# Autodesk Inventor assembly: EL2-.200
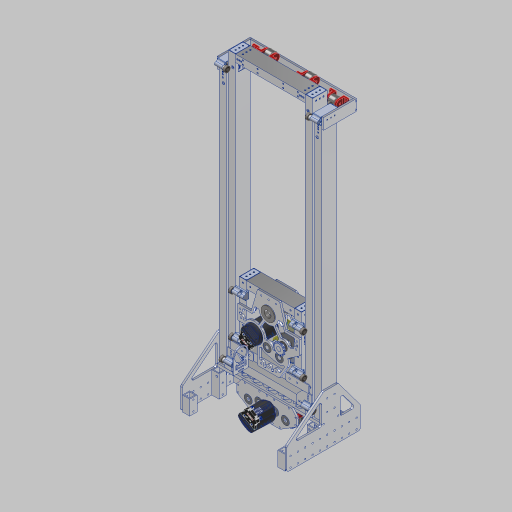
[picture p0: Inventor's stored thumbnail of the model, 512x512]
Saved by Autodesk Inventor 2023.5 (Build 275446000, 446)
## iProperties
Created: 2025-01-11
Part Number: EL2-.200
Document SubType Name: Assembly
Designer: slick
Author: slick
## Documents named in this file (17)
- C:\Users\slick\OneDrive\Desktop\2025-ReefScape---CAD\Elevator\EL2\EL2-.200.iam
- C:\Users\slick\OneDrive\Desktop\2025-ReefScape---CAD\Elevator\EL2\EL2-003.ipt
- C:\Users\slick\OneDrive\Desktop\2025-ReefScape---CAD\Elevator\EL2\EL2-.100.iam
- C:\Users\slick\OneDrive\Desktop\2025-ReefScape---CAD\Elevator\EL2\EL2-.300.iam
- C:\Users\slick\OneDrive\Desktop\2025-ReefScape---CAD\Elevator\EL2\EL2-C-100.iam
- C:\Users\slick\OneDrive\Desktop\2025-ReefScape---CAD\Elevator\EL2\EL2-013.ipt
- C:\Users\slick\OneDrive\Desktop\2025-ReefScape---CAD\Elevator\EL2\EL2-S-002.ipt
- C:\Users\slick\OneDrive\Desktop\2025-ReefScape---CAD\Elevator\EL2\EL2-S-003.ipt
- C:\Users\slick\OneDrive\Desktop\2025-ReefScape---CAD\Elevator\EL2\EL2-S-004.ipt
- C:\Users\slick\OneDrive\Desktop\2025-ReefScape---CAD\Elevator\EL2\EL2-400A.iam
- C:\Users\slick\OneDrive\Desktop\2025-ReefScape---CAD\Elevator\EL2-GB\EL2-GB-100.iam
- C:\Users\slick\OneDrive\Desktop\2025-ReefScape---CAD\Elevator\EL2\EL2-500.iam
- C:\Users\slick\OneDrive\Desktop\2025-ReefScape---CAD\Elevator\EL2\EL2-014.ipt
- C:\Users\slick\OneDrive\Desktop\2025-ReefScape---CAD\Elevator\EL2\EL2-012.ipt
- C:\Users\slick\OneDrive\Desktop\2025-ReefScape---CAD\Elevator\EL2\EL2-600.iam
- C:\Users\slick\OneDrive\Desktop\2025-ReefScape---CAD\Elevator\EL2\EL2-700.iam
- C:\Users\slick\OneDrive\Desktop\2025-ReefScape---CAD\Elevator\EL2\EL2-017.ipt
## Components (30 placed, 16 different names)
1. EL2-003:1 — Mate:3, Mate:7, Mate:8, Mate:9, Mate:10, Insert:41, Insert:42, Insert:47, Insert:64, Insert:65, Insert:66, Insert:67
2. EL2-.100:1 [sub-assembly] — Symmetry:1, Mate:2, Insert:19, Insert:22, Mate:10, Mate:11, Insert:43, Insert:44
3. EL2-.100:2 [sub-assembly] — Symmetry:1, Insert:20, Insert:21, Mate:8, Mate:9, Mate:13, Insert:45, Insert:46
4. EL2-.300:1 [sub-assembly] — Mate:1, Mate:2, Mate:3, Flush:18, Mate:15, Flush:17, Insert:50, Insert:51, Insert:60, Insert:61, Insert:62, Insert:63
5. EL2-C-100:1 [sub-assembly] — Flush:18, Mate:15, Flush:17
6. EL2-013:1 — Insert:48, Insert:49, Insert:56, Insert:57, Insert:58, Insert:59
7. EL2-S-002:1 — Insert:20, Insert:21, Mate:7, Insert:25, Insert:26, Insert:29, Insert:30, Insert:35, Insert:36, Insert:37, Insert:38
8. EL2-S-002:2 — Insert:19, Insert:22, Insert:23, Insert:24, Insert:27, Insert:28, Insert:31, Insert:32, Insert:33, Insert:34, Insert:47
9. EL2-S-003:1 — Insert:25, Insert:26
10. EL2-S-003:2 — Insert:23, Insert:24
11. EL2-S-003:3 — Insert:29, Insert:30
12. EL2-S-003:4 — Insert:27, Insert:28
13. EL2-S-004:1 — Insert:33, Insert:34, Mate:12
14. EL2-S-004:2 — Insert:31, Insert:32
15. EL2-S-004:3 — Insert:35, Insert:36, Mate:14
16. EL2-S-004:4 — Insert:37, Insert:38
17. EL2-400A:1 [sub-assembly] — Mate:11, Mate:12
18. EL2-400A:2 [sub-assembly] — Mate:13, Mate:14
19. EL2-GB-100:1 [sub-assembly] — Insert:41, Insert:42
20. EL2-500:1 [sub-assembly]
21. EL2-014:1 — Insert:43, Insert:44, Insert:48, Insert:49
22. EL2-014:2 — Insert:45, Insert:46
23. EL2-012:1 — Insert:50
24. EL2-012:2 — Insert:51
25. EL2-600:1 [sub-assembly] — Insert:56, Insert:57
26. EL2-600:2 [sub-assembly] — Insert:58, Insert:59
27. EL2-700:1 [sub-assembly] — Insert:60, Insert:61
28. EL2-700:2 [sub-assembly] — Insert:62, Insert:63
29. EL2-017:1 — Insert:64, Insert:65
30. EL2-017:2 — Insert:66, Insert:67
## Relationships (58: Insert 43, Mate 12, Flush 2, Symmetry 1)
- Symmetry:1: EL2-.100:1 ↔ EL2-.100:2
- Mate:1: EL2-.300:1
- Mate:2: EL2-.100:1 ↔ EL2-.300:1
- Mate:3: EL2-003:1 ↔ EL2-.300:1
- Flush:18: EL2-.300:1 ↔ EL2-C-100:1
- Insert:19: EL2-.100:1 ↔ EL2-S-002:2
- Insert:20: EL2-.100:2 ↔ EL2-S-002:1
- Insert:21: EL2-.100:2 ↔ EL2-S-002:1
- Insert:22: EL2-.100:1 ↔ EL2-S-002:2
- Mate:7: EL2-003:1 ↔ EL2-S-002:1
- Mate:8: EL2-003:1 ↔ EL2-.100:2
- Mate:9: EL2-003:1 ↔ EL2-.100:2
- Mate:10: EL2-003:1 ↔ EL2-.100:1
- Insert:23: EL2-S-002:2 ↔ EL2-S-003:2
- Insert:24: EL2-S-002:2 ↔ EL2-S-003:2
- Insert:25: EL2-S-002:1 ↔ EL2-S-003:1
- Insert:26: EL2-S-002:1 ↔ EL2-S-003:1
- Insert:27: EL2-S-002:2 ↔ EL2-S-003:4
- Insert:28: EL2-S-002:2 ↔ EL2-S-003:4
- Insert:29: EL2-S-002:1 ↔ EL2-S-003:3
- Insert:30: EL2-S-002:1 ↔ EL2-S-003:3
- Insert:31: EL2-S-002:2 ↔ EL2-S-004:2
- Insert:32: EL2-S-002:2 ↔ EL2-S-004:2
- Insert:33: EL2-S-002:2 ↔ EL2-S-004:1
- Insert:34: EL2-S-002:2 ↔ EL2-S-004:1
- Insert:35: EL2-S-002:1 ↔ EL2-S-004:3
- Insert:36: EL2-S-002:1 ↔ EL2-S-004:3
- Mate:11: EL2-.100:1 ↔ EL2-400A:1
- Mate:12: EL2-S-004:1 ↔ EL2-400A:1
- Mate:13: EL2-.100:2 ↔ EL2-400A:2
- Mate:14: EL2-S-004:3 ↔ EL2-400A:2
- Insert:37: EL2-S-002:1 ↔ EL2-S-004:4
- Insert:38: EL2-S-002:1 ↔ EL2-S-004:4
- Mate:15: EL2-.300:1 ↔ EL2-C-100:1
- Flush:17: EL2-.300:1 ↔ EL2-C-100:1
- Insert:41: EL2-003:1 ↔ EL2-GB-100:1
- Insert:42: EL2-003:1 ↔ EL2-GB-100:1
- Insert:43: EL2-.100:1 ↔ EL2-014:1
- Insert:44: EL2-.100:1 ↔ EL2-014:1
- Insert:45: EL2-.100:2 ↔ EL2-014:2
- Insert:46: EL2-.100:2 ↔ EL2-014:2
- Insert:47: EL2-003:1 ↔ EL2-S-002:2
- Insert:48: EL2-013:1 ↔ EL2-014:1
- Insert:49: EL2-013:1 ↔ EL2-014:1
- Insert:50: EL2-.300:1 ↔ EL2-012:1
- Insert:51: EL2-.300:1 ↔ EL2-012:2
- Insert:56: EL2-013:1 ↔ EL2-600:1
- Insert:57: EL2-013:1 ↔ EL2-600:1
- Insert:58: EL2-013:1 ↔ EL2-600:2
- Insert:59: EL2-013:1 ↔ EL2-600:2
- Insert:60: EL2-.300:1 ↔ EL2-700:1
- Insert:61: EL2-.300:1 ↔ EL2-700:1
- Insert:62: EL2-.300:1 ↔ EL2-700:2
- Insert:63: EL2-.300:1 ↔ EL2-700:2
- Insert:64: EL2-003:1 ↔ EL2-017:1
- Insert:65: EL2-003:1 ↔ EL2-017:1
- Insert:66: EL2-003:1 ↔ EL2-017:2
- Insert:67: EL2-003:1 ↔ EL2-017:2
